# Autodesk Inventor assembly: still pipe
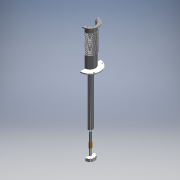
[picture p0: Inventor's stored thumbnail of the model, 180x180]
Saved by Autodesk Inventor 2018 (Build 220112000, 112)
## iProperties
Created: 2019-01-14
Part Number: still pipe
Document SubType Name: Assembly
Designer: Admin
Author: Admin
## Documents named in this file (8)
- C:\Users\Admin\Documents\Cryostat\CAD\still pipe.iam
- C:\Users\Admin\Documents\Cryostat\CAD\KF50 bellows.ipt
- C:\Users\Admin\Documents\Cryostat\CAD\universal connector.ipt
- C:\Users\Admin\Documents\Cryostat\CAD\1in ss pipe.ipt
- C:\Users\Admin\Documents\Cryostat\CAD\0in5 ss pipe.ipt
- C:\Users\Admin\Documents\Cryostat\CAD\adapter.ipt
- C:\Users\Admin\Documents\Cryostat\CAD\heatsink.ipt
- C:\Users\Admin\Documents\Cryostat\CAD\brassbushing2.ipt
## Components (7 placed, 7 different names)
1. KF50 bellows:1 — Mate:16, Flush:2
2. universal connector:1 — Mate:21, Mate:24
3. 1in ss pipe:3 — Mate:15, Flush:1, Mate:17, Mate:23
4. 0in5 ss pipe:1 — Mate:20, Mate:23, Mate:25
5. adapter:1 — Mate:15, Flush:1, Mate:16, Flush:2, Mate:18, Mate:19
6. heatsink:1 — Mate:17, Mate:18, Mate:19, Mate:22
7. brassbushing2:1 — Mate:20, Mate:21, Mate:24, Mate:25
## Relationships (13: Mate 11, Flush 2)
- Mate:15: 1in ss pipe:3 ↔ adapter:1
- Flush:1: 1in ss pipe:3 ↔ adapter:1
- Mate:16: KF50 bellows:1 ↔ adapter:1
- Flush:2: KF50 bellows:1 ↔ adapter:1
- Mate:17: 1in ss pipe:3 ↔ heatsink:1
- Mate:18: adapter:1 ↔ heatsink:1
- Mate:19: adapter:1 ↔ heatsink:1
- Mate:20: 0in5 ss pipe:1 ↔ brassbushing2:1
- Mate:21: universal connector:1 ↔ brassbushing2:1
- Mate:22: heatsink:1
- Mate:23: 1in ss pipe:3 ↔ 0in5 ss pipe:1
- Mate:24: universal connector:1 ↔ brassbushing2:1
- Mate:25: 0in5 ss pipe:1 ↔ brassbushing2:1
